# Autodesk Inventor assembly: Z25_Folding_Arm
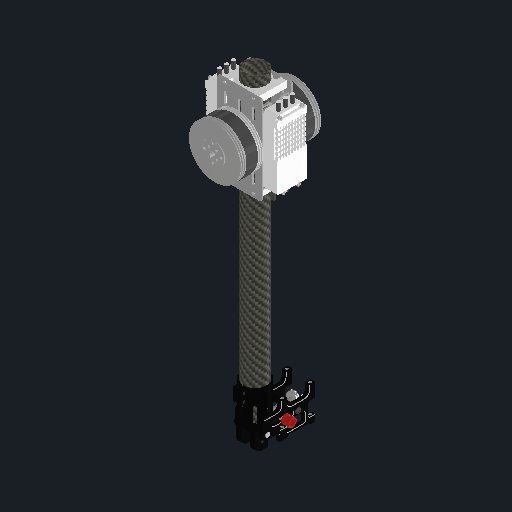
[picture p0: Inventor's stored thumbnail of the model, 512x512]
Saved by Autodesk Inventor 2024.1 (Build 281209000, 209)
## iProperties
Created: 2023-02-14
Part Number: Z25_Folding_Arm
Document SubType Name: Assembly
Designer: dzw04
Author: dzw04
## Documents named in this file (16)
- C:\Users\dzw04\Saxion\Mechatronica Lectoraat LMECH LED - Database ARG\Component_Database\SARAX\01. CAD\01. 3D_Drawing\02. Sub_Assemblies\Z25_Folding_Arm\Old\Z25_Folding_Arm.iam
- C:\Users\dzw04\Saxion\Mechatronica Lectoraat LMECH LED - Database ARG\Component_Database\SARAX\01. CAD\01. 3D_Drawing\02. Sub_Assemblies\Z25_Folding_Arm\01. Parts\Z25_Sideplate.ipt
- C:\Users\dzw04\Saxion\Mechatronica Lectoraat LMECH LED - Database ARG\Component_Database\SARAX\01. CAD\01. 3D_Drawing\02. Sub_Assemblies\Z25_Folding_Arm\01. Parts\Z25_Hinge_Shaft.ipt
- C:\Users\dzw04\Saxion\Mechatronica Lectoraat LMECH LED - Database ARG\Component_Database\SARAX\01. CAD\01. 3D_Drawing\02. Sub_Assemblies\Z25_Folding_Arm\01. Parts\Z25_Spacer.ipt
- C:\Users\dzw04\Saxion\Mechatronica Lectoraat LMECH LED - Database ARG\Component_Database\SARAX\01. CAD\01. 3D_Drawing\02. Sub_Assemblies\Z25_Folding_Arm\01. Parts\Z25_Slide_Spacer.ipt
- C:\Users\dzw04\Saxion\Mechatronica Lectoraat LMECH LED - Database ARG\Component_Database\SARAX\01. CAD\01. 3D_Drawing\02. Sub_Assemblies\Z25_Folding_Arm\01. Parts\Z25_Slide_Shaft.ipt
- C:\Users\dzw04\Saxion\Mechatronica Lectoraat LMECH LED - Database ARG\Component_Database\SARAX\01. CAD\01. 3D_Drawing\02. Sub_Assemblies\Z25_Folding_Arm\01. Parts\Z25_Side_Lock_Button.ipt
- C:\Users\dzw04\Saxion\Mechatronica Lectoraat LMECH LED - Database ARG\Component_Database\SARAX\01. CAD\01. 3D_Drawing\02. Sub_Assemblies\Z25_Folding_Arm\01. Parts\Z25_Pipe_Clamp.ipt
- C:\Users\dzw04\OneDrive - Saxion\Documenten\Inventor\Content Center Files\R2022\en-US\ISO 4762(2)\ISO 4762 - M3 x 8ISO.ipt
- C:\Users\dzw04\OneDrive - Saxion\Documenten\Inventor\Content Center Files\R2022\en-US\ISO 4762(2)\ISO 4762 - M3 x 10ISO.ipt
- C:\Users\dzw04\OneDrive - Saxion\Documenten\Inventor\Content Center Files\R2022\en-US\ISO 7045  H\ISO 7045 - M2,5 x 6_ - 4.8 - H - ISO.ipt
- C:\Users\dzw04\Saxion\Mechatronica Lectoraat LMECH LED - Database ARG\Component_Database\SARAX\01. CAD\01. 3D_Drawing\01. Parts\en-US\ISO 7380-1\ISO 7380-1 - M3 x 6.ipt
- C:\Users\dzw04\OneDrive - Saxion\Documenten\Inventor\Content Center Files\R2022\en-US\DIN 125-1  A\DIN 125 - A 2,7.ipt
- C:\Users\dzw04\Saxion\Mechatronica Lectoraat LMECH LED - Database ARG\Component_Database\SARAX\01. CAD\01. 3D_Drawing\02. Sub_Assemblies\Arm\01. Parts\Tube_25x2x300_CFRP.ipt
- C:\Users\dzw04\Saxion\Mechatronica Lectoraat LMECH LED - Database ARG\Component_Database\SARAX\01. CAD\03. References\01. 3D_Files\Motor mount v12\Motor mount v12.iam
- C:\Users\dzw04\Saxion\Mechatronica Lectoraat LMECH LED - Database ARG\Component_Database\SARAX\01. CAD\01. 3D_Drawing\Parameters.xlsx
## Components (19 placed, 14 different names)
1. Z25_Sideplate:1 — Mate:1, Flush:1, Flush:2, Mate:6, Flush:11, Mate:11, Mate:25, Mate:33, Angle:1
2. Z25_Sideplate:2 — Mate:1, Flush:1, Flush:2, Mate:2, Mate:3, Mate:7, Mate:18, Rotational:1, Mate:31, Flush:12
3. Z25_Hinge_Shaft:1 — Mate:2, Mate:3, Mate:26
4. Z25_Slide_Spacer:1 — Mate:6, Mate:7, Mate:13, Mate:14, Mate:15, Mate:16, Mate:17
5. Z25_Slide_Shaft:1 — Mate:12, Mate:13, Flush:12
6. Z25_Spacer:1 — Flush:11, Mate:11, Mate:12, Mate:32, Mate:34
7. Z25_Side_Lock_Button:1 — Mate:14, Mate:15, Mate:29, Mate:30
8. Z25_Side_Lock_Button:2 — Mate:16, Mate:17, Mate:27, Mate:28
9. Z25_Pipe_Clamp:1 — Mate:18, Rotational:1, Mate:19, Mate:20, Mate:21, Mate:22, Angle:1, Mate:35, Mate:36, Angle:2
10. ISO 4762 M3 x 8:1 — Mate:27, Mate:28
11. ISO 4762 M3 x 8:2 — Mate:29, Mate:30
12. ISO 4762 M3 x 10:1 — Mate:21, Mate:22
13. ISO 4762 M3 x 10:2 — Mate:19, Mate:20
14. ISO 7045 H M2,5 x 6 - 4.8 - H:1 — Mate:23, Mate:24, Mate:26
15. ISO 7380-1 M3 x 6:1 — Mate:33, Mate:34
16. ISO 7380-1 M3 x 6:2 — Mate:31, Mate:32
17. DIN 125-1 A A 2,7:1 — Mate:23, Mate:24, Mate:25
18. Tube_25x2x300_CFRP:1 — Mate:35, Mate:36, Mate:37, Flush:13
19. Motor mount v12:1 [sub-assembly] — Mate:37, Flush:13, Angle:2
## Relationships (40: Mate 32, Flush 5, Angle 2, RevoluteJoint 1)
- Mate:1 (20 mm): Z25_Sideplate:1 ↔ Z25_Sideplate:2
- Flush:1: Z25_Sideplate:1 ↔ Z25_Sideplate:2
- Flush:2: Z25_Sideplate:1 ↔ Z25_Sideplate:2
- Mate:2: Z25_Sideplate:2 ↔ Z25_Hinge_Shaft:1
- Mate:3: Z25_Sideplate:2 ↔ Z25_Hinge_Shaft:1
- Mate:6: Z25_Sideplate:1 ↔ Z25_Slide_Spacer:1
- Mate:7: Z25_Sideplate:2 ↔ Z25_Slide_Spacer:1
- Flush:11 (0.25 mm): Z25_Sideplate:1 ↔ Z25_Spacer:1
- Mate:11: Z25_Sideplate:1 ↔ Z25_Spacer:1
- Mate:12: Z25_Slide_Shaft:1 ↔ Z25_Spacer:1
- Mate:13 (-5 mm): Z25_Slide_Spacer:1 ↔ Z25_Slide_Shaft:1
- Mate:14: Z25_Slide_Spacer:1 ↔ Z25_Side_Lock_Button:1
- Mate:15: Z25_Slide_Spacer:1 ↔ Z25_Side_Lock_Button:1
- Mate:16: Z25_Slide_Spacer:1 ↔ Z25_Side_Lock_Button:2
- Mate:17: Z25_Slide_Spacer:1 ↔ Z25_Side_Lock_Button:2
- Mate:18: Z25_Sideplate:2 ↔ Z25_Pipe_Clamp:1
- Rotational:1 [RevoluteJoint]: Z25_Sideplate:2 ↔ Z25_Pipe_Clamp:1
- Mate:19: Z25_Pipe_Clamp:1 ↔ ISO 4762 M3 x 10:2
- Mate:20: Z25_Pipe_Clamp:1 ↔ ISO 4762 M3 x 10:2
- Mate:21: Z25_Pipe_Clamp:1 ↔ ISO 4762 M3 x 10:1
- Mate:22: Z25_Pipe_Clamp:1 ↔ ISO 4762 M3 x 10:1
- Mate:23: ISO 7045 H M2,5 x 6 - 4.8 - H:1 ↔ DIN 125-1 A A 2,7:1
- Mate:24: ISO 7045 H M2,5 x 6 - 4.8 - H:1 ↔ DIN 125-1 A A 2,7:1
- Mate:25: Z25_Sideplate:1 ↔ DIN 125-1 A A 2,7:1
- Mate:26: Z25_Hinge_Shaft:1 ↔ ISO 7045 H M2,5 x 6 - 4.8 - H:1
- Mate:27: Z25_Side_Lock_Button:2 ↔ ISO 4762 M3 x 8:1
- Mate:28: Z25_Side_Lock_Button:2 ↔ ISO 4762 M3 x 8:1
- Mate:29: Z25_Side_Lock_Button:1 ↔ ISO 4762 M3 x 8:2
- Mate:30: Z25_Side_Lock_Button:1 ↔ ISO 4762 M3 x 8:2
- Mate:31: Z25_Sideplate:2 ↔ ISO 7380-1 M3 x 6:2
- Mate:32: Z25_Spacer:1 ↔ ISO 7380-1 M3 x 6:2
- Mate:33: Z25_Sideplate:1 ↔ ISO 7380-1 M3 x 6:1
- Mate:34: Z25_Spacer:1 ↔ ISO 7380-1 M3 x 6:1
- Angle:1 (-90 deg): Z25_Sideplate:1 ↔ Z25_Pipe_Clamp:1
- Flush:12: Z25_Sideplate:2 ↔ Z25_Slide_Shaft:1
- Mate:35: Z25_Pipe_Clamp:1 ↔ Tube_25x2x300_CFRP:1
- Mate:36: Z25_Pipe_Clamp:1 ↔ Tube_25x2x300_CFRP:1
- Mate:37: Tube_25x2x300_CFRP:1 ↔ Motor mount v12:1
- Flush:13 (10 mm): Tube_25x2x300_CFRP:1 ↔ Motor mount v12:1
- Angle:2 (0 deg): Z25_Pipe_Clamp:1 ↔ Motor mount v12:1
## Named parameters: BatteryLength = 200 mm, BatteryWidth = 62 mm, BatteryHeight = 76 mm, NumberOfArms = 4, RotorToRotor = 900 mm, MountToMotorCenter = 0 mm, ArmPosition = 90 deg, ThicknessBodyCenterPlate = 2 mm, ThicknessBodyOuterPlate = 2 mm, ThicknessLegLoadpipePlate = 2 mm, ThicknessBatteryTray = 2 mm, ThicknessBatteryTopTray = 1 mm, LoadpipeLength = 450 mm, NumberOfBatterys = 2, LandingGearHeight = 400 mm, LandingGearStabilityBar = 525 mm, LandingGearRod = 390 mm
